# Autodesk Inventor assembly: lightweight carrige v2
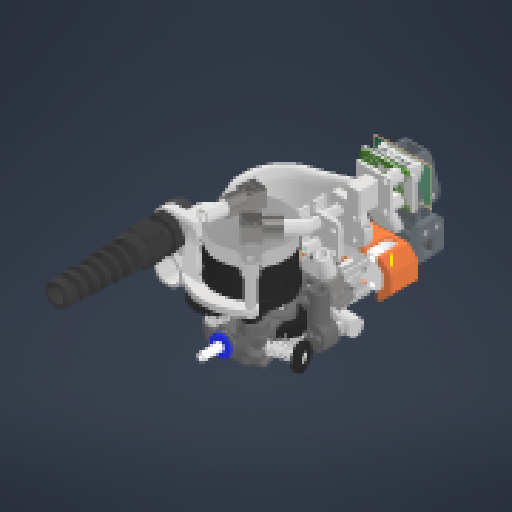
[picture p0: Inventor's stored thumbnail of the model, 512x512]
Saved by Autodesk Inventor 2024.3 (Build 283343010, 343A)
## iProperties
Created: 2024-09-28
Part Number: lightweight carrige v2
Document SubType Name: Assembly
Designer: MFil
Mass: 257.971 g
Surface Area: 556.316 cm^2
Volume: 46.6137 cm^3
Density: 5.53423 g/cm^3
Author: MFil
## Documents named in this file (33)
- C:\ROBOTYKA\myVORON-tridex\Hotend carriges\lightweight carrige v2 PROTOX TRY.iam
- C:\ROBOTYKA\myVORON-tridex\Hotend carriges\thin carrige\MGN9H Block.ipt
- C:\ROBOTYKA\myVORON-tridex\Hotend carriges\thin carrige\LDO-36STH20-1004AHG.ipt
- C:\ROBOTYKA\myVORON-tridex\Hotend carriges\thin carrige\LGX 17T-44T Gear.ipt
- C:\ROBOTYKA\myVORON-tridex\Hotend carriges\thin carrige\LGX Hobbed Gear (R).iam
- C:\ROBOTYKA\myVORON-tridex\Hotend carriges\thin carrige\MR63ZZ (B).ipt
- C:\ROBOTYKA\myVORON-tridex\Hotend carriges\thin carrige\Rocker shaft.ipt
- C:\ROBOTYKA\myVORON-tridex\Hotend carriges\thin carrige\Rocker screw BASE.iam
- C:\ROBOTYKA\myVORON-tridex\Parts\tridex belt a_CPY 4.ipt
- C:\ROBOTYKA\myVORON-tridex\Hotend carriges\parts\filament piece.ipt
- C:\ROBOTYKA\myVORON-tridex\Hotend carriges\thin carrige\Screw M3x25.ipt
- C:\ROBOTYKA\myVORON-tridex\Hotend carriges\parts\6mm hose fitting.ipt
- C:\ROBOTYKA\myVORON-tridex\Hotend carriges\parts\ptfe filament guide.ipt
- C:\ROBOTYKA\myVORON-tridex\Hotend carriges\parts\colle ptfe guide.ipt
- C:\ROBOTYKA\myVORON-tridex\Hotend carriges\parts\mounting plate.ipt
- C:\ROBOTYKA\myVORON-tridex\Hotend carriges\water hotend v2 assembly.iam
- C:\ROBOTYKA\myVORON-tridex\Parts\PG7 Flex Gland\PG7 Flex Gland\PG7 Flex Gland.iam
- C:\ROBOTYKA\myVORON-tridex\Hotend carriges\20x5 mm spacer.ipt
- C:\ROBOTYKA\myVORON-tridex\Hotend carriges\parts\nema 14 heatsink.ipt
- C:\ROBOTYKA\myVORON-tridex\Hotend carriges\parts\nema 14 cooler lid.ipt
- C:\ROBOTYKA\myVORON-tridex\Hotend carriges\thin carrige\clicky pcb top.ipt
- C:\ROBOTYKA\myVORON-tridex\Hotend carriges\thin carrige\Clicku pcb bottom.ipt
- C:\ROBOTYKA\myVORON-tridex\Hotend carriges\thin carrige\Part2.ipt
- C:\ROBOTYKA\myVORON-tridex\Extruders\ProtoXtruder_HGX_gears\ProtoXtruder_HGX_gears\Idler_arm.ipt
- C:\ROBOTYKA\myVORON-tridex\Extruders\ProtoXtruder_HGX_gears\ProtoXtruder_HGX_gears\Back.ipt
- C:\ROBOTYKA\myVORON-tridex\Hotend carriges\parts\pm6m6 fitting dtraight.ipt
- C:\ROBOTYKA\myVORON-tridex\Hotend carriges\parts\m3x5 35mm standoff.ipt
- C:\ROBOTYKA\myVORON-tridex\Hotend carriges\parts\Klicky-00 - RC2 Assemblies\Klicky-00 - RC2 Assemblies\Klicky-00 - RC2 Assemblies.iam
- C:\ROBOTYKA\myVORON-tridex\Parts\umbilical mount.ipt
- C:\ROBOTYKA\myVORON-tridex\Parts\belt holder xy.ipt
- C:\ROBOTYKA\myVORON-tridex\Parts\belt holder opposite.ipt
- C:\ROBOTYKA\myVORON-tridex\Parts\belt holder 3d printed spacer.ipt
- C:\ROBOTYKA\myVORON-tridex\step files\ProtoXtruder_HGX_gears\ProtoXtruder_HGX_gears\Front_ECAS04.ipt
## Components (39 placed, 32 different names)
1. mounting plate:1 — Flush:28, Mate:54, Mate:55, Mate:84, Flush:114, Mate:164, Mate:165, Mate:166, Flush:115, Mate:173, Mate:174, Mate:189, Mate:190, Mate:191
2. MGN9H Block:1 — Mate:36, Flush:28, Flush:30, Mate:54, Mate:55, Mate:180
3. Rocker shaft:1 — Mate:129
4. Rocker screw BASE:1 [sub-assembly] — Mate:130, Mate:131
5. tridex belt a_CPY 4:1 — Mate:185
6. tridex belt a_CPY 4:2 — Mate:36, Flush:30
7. filament piece:1 — Mate:46, Mate:148
8. LDO-36STH20-1004AHG:1 — Flush:53, Mate:142, Mate:143, Mate:154, Mate:155, Mate:163, Mate:167, Flush:122, Flush:123
9. MR63ZZ (B):1 — Mate:40, Flush:25
10. LGX 17T-44T Gear:1 — Mate:41, Flush:24, Flush:25
11. MR63ZZ (B):2 — Mate:40, Mate:41, Flush:24, Mate:141
12. 6mm hose fitting:1 — Mate:161, Mate:179
13. ptfe filament guide:1 — Mate:85, Mate:148
14. colle ptfe guide:1 — Mate:46
15. 6mm hose fitting:3 — Flush:36
16. 6mm hose fitting:4 — Flush:36, Mate:126
17. water hotend v2 assembly:1 [sub-assembly] — Mate:84, Mate:85, Mate:145, Mate:161, Mate:169, Flush:117, Flush:118, Mate:173, Mate:174, Flush:120, Mate:178, Mate:179
18. PG7 Flex Gland:1 [sub-assembly] — Mate:180, Tangent:16, Flush:124, Tangent:17, Mate:181
19. nema 14 heatsink:1 — Flush:53, Mate:88, Mate:119, Mate:120, Mate:154, Mate:155, Mate:157, Mate:159
20. nema 14 cooler lid:1 — Mate:88, Mate:119, Mate:120, Mate:126, Mate:150
21. clicky pcb top:1 — Mate:170, Mate:171, Flush:116, Mate:175, Mate:176, Mate:177, Flush:121
22. Clicku pcb bottom:1 — Mate:175, Mate:176, Mate:177
23. Part2:1 — Flush:115, Flush:119, Flush:121
24. LGX Hobbed Gear (R):1 [sub-assembly] — Flush:110, Mate:192
25. LGX Hobbed Gear (R):2 [sub-assembly] — Mate:128, Flush:109, Flush:110
26. Idler_arm — Mate:128, Flush:109, Mate:129, Mate:130, Mate:131
27. Back — Mate:141, Mate:142, Mate:143, Mate:163, Mate:193, Mate:194
28. Screw M3x25:6 — Mate:150, Mate:156, Mate:182
29. pm6m6 fitting dtraight:1 — Mate:145, Mate:178
30. 20x5 mm spacer:1 — Mate:156, Mate:157
31. 20x5 mm spacer:2 — Mate:159, Mate:167
32. m3x5 35mm standoff:1 — Flush:114, Mate:165, Mate:183, Mate:186
33. m3x5 35mm standoff:2 — Mate:164, Mate:166, Mate:184, Mate:187
34. Klicky-00 - RC2 Assemblies:1 [sub-assembly] — Mate:169, Mate:170, Mate:171, Flush:116, Flush:117, Flush:118, Flush:119, Flush:120
35. umbilical mount:1 — Flush:122, Flush:123, Tangent:16, Flush:124, Tangent:17, Mate:181, Mate:182
36. belt holder xy:1 — Mate:183, Mate:184, Mate:185, Mate:188
37. belt holder opposite:1 — Mate:186, Mate:187, Mate:188, Flush:125
38. belt holder 3d printed spacer:1 — Flush:125
39. Front_ECAS04:1 — Mate:189, Mate:190, Mate:191, Mate:192, Mate:193, Mate:194
## Relationships (83: Mate 59, Flush 22, Tangent 2)
- [Flush]: tridex belt a_CPY 4:1 ↔ tridex belt a_CPY 4:2
- [Mate] (2.5 mm): tridex belt a_CPY 4:1 ↔ tridex belt a_CPY 4:2
- [Flush]: tridex belt a_CPY 4:1 ↔ tridex belt a_CPY 4:2
- Mate:36 (3.3 mm): MGN9H Block:1 ↔ tridex belt a_CPY 4:2
- Mate:40: MR63ZZ (B):1 ↔ MR63ZZ (B):2
- Mate:41: LGX 17T-44T Gear:1 ↔ MR63ZZ (B):2
- Flush:24: LGX 17T-44T Gear:1 ↔ MR63ZZ (B):2
- Flush:25: MR63ZZ (B):1 ↔ LGX 17T-44T Gear:1
- Mate:46: filament piece:1 ↔ colle ptfe guide:1
- Flush:28: mounting plate:1 ↔ MGN9H Block:1
- Flush:30 (10.831 mm): MGN9H Block:1 ↔ tridex belt a_CPY 4:2
- Mate:54: mounting plate:1 ↔ MGN9H Block:1
- Mate:55: mounting plate:1 ↔ MGN9H Block:1
- Flush:36: 6mm hose fitting:3 ↔ 6mm hose fitting:4
- Mate:84: mounting plate:1 ↔ water hotend v2 assembly:1
- Mate:85: ptfe filament guide:1 ↔ water hotend v2 assembly:1
- Flush:53: LDO-36STH20-1004AHG:1 ↔ nema 14 heatsink:1
- Mate:88: nema 14 heatsink:1 ↔ nema 14 cooler lid:1
- Mate:119: nema 14 heatsink:1 ↔ nema 14 cooler lid:1
- Mate:120: nema 14 heatsink:1 ↔ nema 14 cooler lid:1
- Mate:126: 6mm hose fitting:4 ↔ nema 14 cooler lid:1
- Mate:128: LGX Hobbed Gear (R):2 ↔ Idler_arm
- Flush:109: LGX Hobbed Gear (R):2 ↔ Idler_arm
- Mate:129: Rocker shaft:1 ↔ Idler_arm
- Mate:130: Rocker screw BASE:1 ↔ Idler_arm
- Mate:131: Rocker screw BASE:1 ↔ Idler_arm
- Flush:110: LGX Hobbed Gear (R):1 ↔ LGX Hobbed Gear (R):2
- Mate:141: MR63ZZ (B):2 ↔ Back
- Mate:142: LDO-36STH20-1004AHG:1 ↔ Back
- Mate:143: LDO-36STH20-1004AHG:1 ↔ Back
- Mate:145: water hotend v2 assembly:1 ↔ pm6m6 fitting dtraight:1
- Mate:148: filament piece:1 ↔ ptfe filament guide:1
- Mate:150: nema 14 cooler lid:1 ↔ Screw M3x25:6
- Mate:154: LDO-36STH20-1004AHG:1 ↔ nema 14 heatsink:1
- Mate:155: LDO-36STH20-1004AHG:1 ↔ nema 14 heatsink:1
- Mate:156: Screw M3x25:6 ↔ 20x5 mm spacer:1
- Mate:157: nema 14 heatsink:1 ↔ 20x5 mm spacer:1
- Mate:159: nema 14 heatsink:1 ↔ 20x5 mm spacer:2
- Mate:161: 6mm hose fitting:1 ↔ water hotend v2 assembly:1
- Mate:163: LDO-36STH20-1004AHG:1 ↔ Back
- Flush:114: mounting plate:1 ↔ m3x5 35mm standoff:1
- Mate:164: mounting plate:1 ↔ m3x5 35mm standoff:2
- Mate:165: mounting plate:1 ↔ m3x5 35mm standoff:1
- Mate:166: mounting plate:1 ↔ m3x5 35mm standoff:2
- Mate:167: LDO-36STH20-1004AHG:1 ↔ 20x5 mm spacer:2
- Flush:115: mounting plate:1 ↔ Part2:1
- Mate:169: water hotend v2 assembly:1 ↔ Klicky-00 - RC2 Assemblies:1
- Mate:170: clicky pcb top:1 ↔ Klicky-00 - RC2 Assemblies:1
- Mate:171: clicky pcb top:1 ↔ Klicky-00 - RC2 Assemblies:1
- Flush:116: clicky pcb top:1 ↔ Klicky-00 - RC2 Assemblies:1
- Flush:117: water hotend v2 assembly:1 ↔ Klicky-00 - RC2 Assemblies:1
- Flush:118 (6.474 mm): water hotend v2 assembly:1 ↔ Klicky-00 - RC2 Assemblies:1
- Mate:173: mounting plate:1 ↔ water hotend v2 assembly:1
- Mate:174: mounting plate:1 ↔ water hotend v2 assembly:1
- Flush:119: Part2:1 ↔ Klicky-00 - RC2 Assemblies:1
- Flush:120 (3.977 mm): water hotend v2 assembly:1 ↔ Klicky-00 - RC2 Assemblies:1
- Mate:175: clicky pcb top:1 ↔ Clicku pcb bottom:1
- Mate:176: clicky pcb top:1 ↔ Clicku pcb bottom:1
- Mate:177: clicky pcb top:1 ↔ Clicku pcb bottom:1
- Flush:121: clicky pcb top:1 ↔ Part2:1
- Mate:178: water hotend v2 assembly:1 ↔ pm6m6 fitting dtraight:1
- Mate:179: 6mm hose fitting:1 ↔ water hotend v2 assembly:1
- Flush:122: LDO-36STH20-1004AHG:1 ↔ umbilical mount:1
- Flush:123: LDO-36STH20-1004AHG:1 ↔ umbilical mount:1
- Mate:180 (30 mm): MGN9H Block:1 ↔ PG7 Flex Gland:1
- Tangent:16: PG7 Flex Gland:1 ↔ umbilical mount:1
- Flush:124: PG7 Flex Gland:1 ↔ umbilical mount:1
- Tangent:17 (-0.5 mm): PG7 Flex Gland:1 ↔ umbilical mount:1
- Mate:181: PG7 Flex Gland:1 ↔ umbilical mount:1
- Mate:182: Screw M3x25:6 ↔ umbilical mount:1
- Mate:183: m3x5 35mm standoff:1 ↔ belt holder xy:1
- Mate:184: m3x5 35mm standoff:2 ↔ belt holder xy:1
- Mate:185 (3 mm): tridex belt a_CPY 4:1 ↔ belt holder xy:1
- Mate:186: m3x5 35mm standoff:1 ↔ belt holder opposite:1
- Mate:187: m3x5 35mm standoff:2 ↔ belt holder opposite:1
- Mate:188 (9 mm): belt holder xy:1 ↔ belt holder opposite:1
- Flush:125: belt holder opposite:1 ↔ belt holder 3d printed spacer:1
- Mate:189: mounting plate:1 ↔ Front_ECAS04:1
- Mate:190: mounting plate:1 ↔ Front_ECAS04:1
- Mate:191: mounting plate:1 ↔ Front_ECAS04:1
- Mate:192: LGX Hobbed Gear (R):1 ↔ Front_ECAS04:1
- Mate:193: Back ↔ Front_ECAS04:1
- Mate:194: Back ↔ Front_ECAS04:1
